# Autodesk Inventor assembly: LaptopTopDisplay
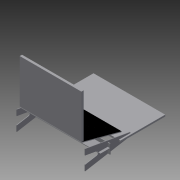
[picture p0: Inventor's stored thumbnail of the model, 180x180]
Saved by Autodesk Inventor 2017 (Build 210142000, 142)
## iProperties
Created: 2019-02-02
Part Number: LaptopTopDisplay
Document SubType Name: Assembly
Designer: ari
Author: ari
## Documents named in this file (5)
- C:\Users\ari\Documents\Inventor\LaptopTopDisplay\LaptopTopDisplay.iam
- C:\Users\ari\Documents\Inventor\LaptopTopDisplay\laptop.ipt
- C:\Users\ari\Documents\Inventor\LaptopTopDisplay\stand.ipt
- C:\Users\ari\Documents\Inventor\LaptopTopDisplay\brace.ipt
- C:\Users\ari\Documents\Inventor\LaptopTopDisplay\extDisplay.ipt
## Components (6 placed, 4 different names)
1. laptop:1 — Flush:3
2. stand:1 — Mate:6, Mate:7, Mate:8, Mate:9, Flush:3
3. stand:2 — Mate:1, Mate:2, Mate:3, Mate:4, Mate:10, Flush:1
4. brace:1 — Mate:3, Mate:4, Mate:5, Mate:6, Mate:7, Flush:2
5. brace:2 — Mate:1, Mate:2, Mate:5, Mate:8, Flush:2
6. extDisplay:1 — Mate:9, Mate:10, Flush:1
## Relationships (13: Mate 10, Flush 3)
- Mate:1 (0.025 mm): stand:2 ↔ brace:2
- Mate:2: stand:2 ↔ brace:2
- Mate:3 (0.025 mm): stand:2 ↔ brace:1
- Mate:4 (0.025 mm): stand:2 ↔ brace:1
- Mate:5 (0.025 mm): brace:1 ↔ brace:2
- Mate:6 (0.025 mm): stand:1 ↔ brace:1
- Mate:7 (0.025 mm): stand:1 ↔ brace:1
- Mate:8 (0.025 mm): stand:1 ↔ brace:2
- Mate:9: stand:1 ↔ extDisplay:1
- Mate:10: stand:2 ↔ extDisplay:1
- Flush:1 (7 mm): stand:2 ↔ extDisplay:1
- Flush:2 (27 mm): brace:1 ↔ brace:2
- Flush:3: laptop:1 ↔ stand:1
## Named parameters: u = 0.05 mm
